# Autodesk Inventor assembly: HK0408FT2
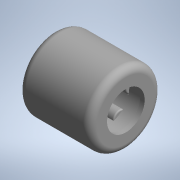
[picture p0: Inventor's stored thumbnail of the model, 180x180]
Saved by Autodesk Inventor 2021 (Build 250183000, 183)
## iProperties
Part Number: HK0408FT2
Catalog Web Link: www.cadenas.de
Description: HK,HK..ZWD,HMK,HMK..ZWD (Open-end)-
Vendor: NTN
Document SubType Name: Assembly
Designer: partserver
Manufacturer: NTN
Mass: 0.214966 g
Surface Area: 8.40255 cm^2
Volume: 0.214966 cm^3
Density: 1 g/cm^3
Category: PARTsolutions
Company: NTN
PSOL_IDENT_0: {$CADENAS_DATA\23d-libs\ntn\needle_roler_bearings\needle_roller_shell_bearings\needle_roller_shell_b
PSOL_IDENT_1: earings_open_ended_asmtab.prj},200 {VTYP=3D},{STYP=ASSTAB},{NB=HK0408FT2},{LINA=HK0408FT2},{NN=HK,HK
PSOL_IDENT_2: ..ZWD,HMK,HMK..ZWD (Open-end)},{DATE=23.10.2020 01:12:41},{GEOMDATE=22.04.2020 01:03:43},{VERSION=},
PSOL_IDENT_3: {LINEID=20},{WBVAR=},{WBNUMERIC=}  {NB=HK0408FT2},{LINA=HK0408FT2},{KT=DUMMY},{ORDER=HK0408FT2},{FW=
PSOL_IDENT_4: 4},{D=8.0},{C=8},{CR=1770},{COR=1270},{CU=155},{CRF=180},{CORF=129},{LSG=30000},{LSO=45000},{MASS=0.
PSOL_IDENT_5: 0016},{IT=-},{RT=1.6},{VER=1},{T=0.500},{DW=1.500},{LW=4.000},{NR=6.000},{CID=4.750},{CD=6.250},{CW=
PSOL_IDENT_6: 6.600},{SD=4.200},{PPATH=../needle_roller_shell_bearings_open_ended_asmtpl.prj}
NB: HK0408FT2
NN: HK,HK..ZWD,HMK,HMK..ZWD (Open-end)
NBSYN: $ORDER.
LINA: HK0408FT2
CATALOG: NTN Corporation
ORDER: HK0408FT2
FW: 4
D: 8
C: 8
CR: 1770
COR: 1270
CU: 155
LSG: 30000
LSO: 45000
MASS: 0.0016
IT: -
SUPPLIER: NTN
ARTICLENO: HK0408FT2
BOMINFO: HK0408FT2
CREATOR: CADENAS GmbH
Title: HK0408FT2
Author: Cadenas PARTsolutions
## Documents named in this file (4)
- C:\Users\YusukeKunita\Documents\GrabCAD\NHK2021\BasicParts\よく使う部品（萩原）\Bearing\Bearing_HK0408T2\HK0408FT2.iam
- C:\Users\YusukeKunita\Documents\GrabCAD\NHK2021\BasicParts\よく使う部品（萩原）\Bearing\Bearing_HK0408T2\HK0408FT2SH.ipt
- C:\Users\YusukeKunita\Documents\GrabCAD\NHK2021\BasicParts\よく使う部品（萩原）\Bearing\Bearing_HK0408T2\HK0408FT2CA.ipt
- C:\Users\YusukeKunita\Documents\GrabCAD\NHK2021\BasicParts\よく使う部品（萩原）\Bearing\Bearing_HK0408T2\HK0408FT2RO.ipt
## Components (8 placed, 3 different names)
1. HK0408FT2SH:1 — IP_5_XY@1 <-> IP_1_XY@2, IP_5_Z@1 <-> IP_1_Z@2
2. HK0408FT2CA:1 — IP_5_XY@1 <-> IP_1_XY@2, IP_5_Z@1 <-> IP_1_Z@2, IP_3_1_XY@2 <-> IP_1_XY@3, IP_3_1_Z@2 <-> IP_1_Z@3, IP_3_1_YZ@2 <-> IP_1_YZ@3, IP_3_2_XY@2 <-> IP_1_XY@4, IP_3_2_Z@2 <-> IP_1_Z@4, IP_3_2_YZ@2 <-> IP_1_YZ@4, IP_3_3_XY@2 <-> IP_1_XY@5, IP_3_3_Z@2 <-> IP_1_Z@5, IP_3_3_YZ@2 <-> IP_1_YZ@5, IP_3_4_XY@2 <-> IP_1_XY@6, IP_3_4_Z@2 <-> IP_1_Z@6, IP_3_4_YZ@2 <-> IP_1_YZ@6, IP_3_5_XY@2 <-> IP_1_XY@7, IP_3_5_Z@2 <-> IP_1_Z@7, IP_3_5_YZ@2 <-> IP_1_YZ@7, IP_3_6_XY@2 <-> IP_1_XY@8, IP_3_6_Z@2 <-> IP_1_Z@8, IP_3_6_YZ@2 <-> IP_1_YZ@8
3. HK0408FT2RO:1 — IP_3_1_XY@2 <-> IP_1_XY@3, IP_3_1_Z@2 <-> IP_1_Z@3, IP_3_1_YZ@2 <-> IP_1_YZ@3
4. HK0408FT2RO:2 — IP_3_2_XY@2 <-> IP_1_XY@4, IP_3_2_Z@2 <-> IP_1_Z@4, IP_3_2_YZ@2 <-> IP_1_YZ@4
5. HK0408FT2RO:3 — IP_3_3_XY@2 <-> IP_1_XY@5, IP_3_3_Z@2 <-> IP_1_Z@5, IP_3_3_YZ@2 <-> IP_1_YZ@5
6. HK0408FT2RO:4 — IP_3_4_XY@2 <-> IP_1_XY@6, IP_3_4_Z@2 <-> IP_1_Z@6, IP_3_4_YZ@2 <-> IP_1_YZ@6
7. HK0408FT2RO:5 — IP_3_5_XY@2 <-> IP_1_XY@7, IP_3_5_Z@2 <-> IP_1_Z@7, IP_3_5_YZ@2 <-> IP_1_YZ@7
8. HK0408FT2RO:6 — IP_3_6_XY@2 <-> IP_1_XY@8, IP_3_6_Z@2 <-> IP_1_Z@8, IP_3_6_YZ@2 <-> IP_1_YZ@8
## Relationships (20: Mate 13, Angle 6, Flush 1)
- IP_5_XY@1 <-> IP_1_XY@2 [Flush]: HK0408FT2SH:1 ↔ HK0408FT2CA:1
- IP_5_Z@1 <-> IP_1_Z@2 [Mate]: HK0408FT2SH:1 ↔ HK0408FT2CA:1
- IP_3_1_XY@2 <-> IP_1_XY@3 [Mate]: HK0408FT2CA:1 ↔ HK0408FT2RO:1
- IP_3_1_Z@2 <-> IP_1_Z@3 [Mate]: HK0408FT2CA:1 ↔ HK0408FT2RO:1
- IP_3_1_YZ@2 <-> IP_1_YZ@3 [Angle] (0 deg): HK0408FT2CA:1 ↔ HK0408FT2RO:1
- IP_3_2_XY@2 <-> IP_1_XY@4 [Mate]: HK0408FT2CA:1 ↔ HK0408FT2RO:2
- IP_3_2_Z@2 <-> IP_1_Z@4 [Mate]: HK0408FT2CA:1 ↔ HK0408FT2RO:2
- IP_3_2_YZ@2 <-> IP_1_YZ@4 [Angle] (0 deg): HK0408FT2CA:1 ↔ HK0408FT2RO:2
- IP_3_3_XY@2 <-> IP_1_XY@5 [Mate]: HK0408FT2CA:1 ↔ HK0408FT2RO:3
- IP_3_3_Z@2 <-> IP_1_Z@5 [Mate]: HK0408FT2CA:1 ↔ HK0408FT2RO:3
- IP_3_3_YZ@2 <-> IP_1_YZ@5 [Angle] (0 deg): HK0408FT2CA:1 ↔ HK0408FT2RO:3
- IP_3_4_XY@2 <-> IP_1_XY@6 [Mate]: HK0408FT2CA:1 ↔ HK0408FT2RO:4
- IP_3_4_Z@2 <-> IP_1_Z@6 [Mate]: HK0408FT2CA:1 ↔ HK0408FT2RO:4
- IP_3_4_YZ@2 <-> IP_1_YZ@6 [Angle] (0 deg): HK0408FT2CA:1 ↔ HK0408FT2RO:4
- IP_3_5_XY@2 <-> IP_1_XY@7 [Mate]: HK0408FT2CA:1 ↔ HK0408FT2RO:5
- IP_3_5_Z@2 <-> IP_1_Z@7 [Mate]: HK0408FT2CA:1 ↔ HK0408FT2RO:5
- IP_3_5_YZ@2 <-> IP_1_YZ@7 [Angle] (0 deg): HK0408FT2CA:1 ↔ HK0408FT2RO:5
- IP_3_6_XY@2 <-> IP_1_XY@8 [Mate]: HK0408FT2CA:1 ↔ HK0408FT2RO:6
- IP_3_6_Z@2 <-> IP_1_Z@8 [Mate]: HK0408FT2CA:1 ↔ HK0408FT2RO:6
- IP_3_6_YZ@2 <-> IP_1_YZ@8 [Angle] (0 deg): HK0408FT2CA:1 ↔ HK0408FT2RO:6
